# Autodesk Inventor assembly: RadLWL
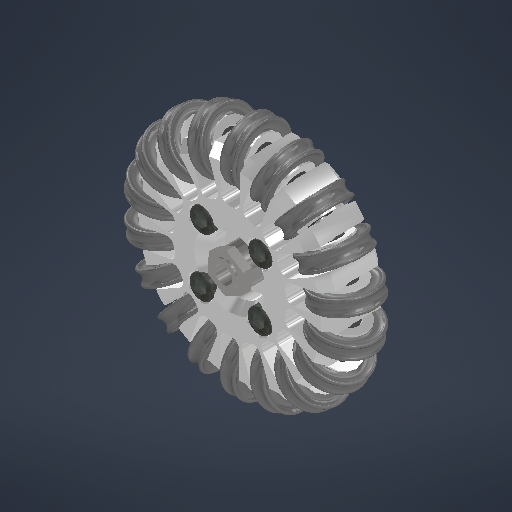
[picture p0: Inventor's stored thumbnail of the model, 512x512]
Saved by Autodesk Inventor 2025.2 (Build 292293000, 293)
## iProperties
Created: 2025-03-24
Part Number: RadLWL
Document SubType Name: Assembly
Designer: Faabs
Author: Faabs
## Documents named in this file (6)
- C:\Users\Faabs\Nextcloud\technulgy\RadLWL\RadLWL.iam
- C:\Users\Faabs\Nextcloud\technulgy\RadLWL\Radkasten.ipt
- C:\Users\Faabs\Nextcloud\technulgy\RadLWL\Rolle\UBG-Rolle.iam
- C:\Users\Faabs\Nextcloud\technulgy\RadLWL\Raddeckel.ipt
- C:\Users\Faabs\Nextcloud\technulgy\RadLWL\Spannsatz\Spannsatz - Bohrung 4mm.iam
- C:\Users\Faabs\Nextcloud\technulgy\RadLWL\DIN 912 - M3 x 0,5 x 6 x 4,75.ipt
## Components (25 placed, 5 different names)
1. Spannsatz - Bohrung 4mm:1 [sub-assembly] — Passend:6, Fluchtend:4
2. Radkasten:1 — Fluchtend:1, Fluchtend:2, Fluchtend:3, Passend:1, Passend:2, Passend:4, Passend:5, Passend:6, Fluchtend:4, Passend:7, Passend:8
3. Raddeckel:1 — Passend:4, Passend:5, Passend:8, Einfügen:1, Einfügen:2, Einfügen:3, Einfügen:4
4. DIN 912 - ersetzt durch DIN EN ISO 4762 M3 x 6:4 — Einfügen:1
5. DIN 912 - ersetzt durch DIN EN ISO 4762 M3 x 6:3 — Einfügen:3
6. DIN 912 - ersetzt durch DIN EN ISO 4762 M3 x 6:2 — Einfügen:4
7. DIN 912 - ersetzt durch DIN EN ISO 4762 M3 x 6:1 — Einfügen:2
8. UBG-Rolle:1 [sub-assembly] — Passend:1, Passend:2, Passend:7
9. UBG-Rolle:2 [sub-assembly]
10. UBG-Rolle:3 [sub-assembly]
11. UBG-Rolle:4 [sub-assembly]
12. UBG-Rolle:5 [sub-assembly]
13. UBG-Rolle:6 [sub-assembly]
14. UBG-Rolle:7 [sub-assembly]
15. UBG-Rolle:8 [sub-assembly]
16. UBG-Rolle:9 [sub-assembly]
17. UBG-Rolle:10 [sub-assembly]
18. UBG-Rolle:11 [sub-assembly]
19. UBG-Rolle:12 [sub-assembly]
20. UBG-Rolle:13 [sub-assembly]
21. UBG-Rolle:14 [sub-assembly]
22. UBG-Rolle:15 [sub-assembly]
23. UBG-Rolle:16 [sub-assembly]
24. UBG-Rolle:17 [sub-assembly]
25. UBG-Rolle:18 [sub-assembly]
## Component patterns: (18 elements, first: UBG-Rolle:1)
## Relationships (15: Mate 7, Flush 4, Insert 4)
- Fluchtend:1 [Flush]: Radkasten:1
- Fluchtend:2 [Flush]: Radkasten:1
- Fluchtend:3 [Flush]: Radkasten:1
- Passend:1 [Mate]: Radkasten:1 ↔ UBG-Rolle:1
- Passend:2 [Mate] (0.2 mm): Radkasten:1 ↔ UBG-Rolle:1
- Passend:4 [Mate]: Radkasten:1 ↔ Raddeckel:1
- Passend:5 [Mate]: Radkasten:1 ↔ Raddeckel:1
- Passend:6 [Mate]: Spannsatz - Bohrung 4mm:1 ↔ Radkasten:1
- Fluchtend:4 [Flush]: Spannsatz - Bohrung 4mm:1 ↔ Radkasten:1
- Passend:7 [Mate] (7 mm): Radkasten:1 ↔ UBG-Rolle:1
- Passend:8 [Mate]: Radkasten:1 ↔ Raddeckel:1
- Einfügen:1 [Insert]: Raddeckel:1 ↔ DIN 912 - ersetzt durch DIN EN ISO 4762 M3 x 6:4
- Einfügen:2 [Insert]: Raddeckel:1 ↔ DIN 912 - ersetzt durch DIN EN ISO 4762 M3 x 6:1
- Einfügen:3 [Insert]: Raddeckel:1 ↔ DIN 912 - ersetzt durch DIN EN ISO 4762 M3 x 6:3
- Einfügen:4 [Insert]: Raddeckel:1 ↔ DIN 912 - ersetzt durch DIN EN ISO 4762 M3 x 6:2
